# Autodesk Inventor assembly: Stadio7
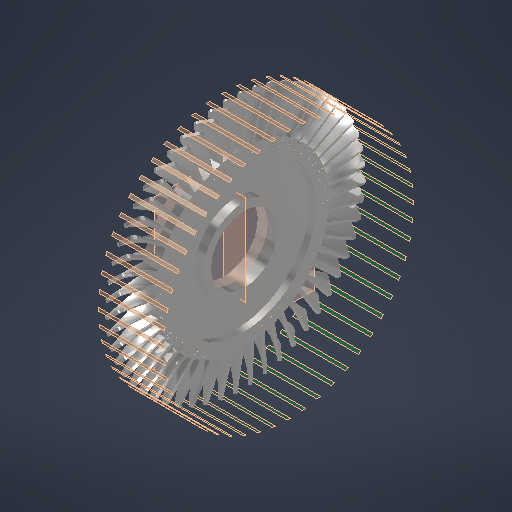
[picture p0: Inventor's stored thumbnail of the model, 512x512]
Saved by Autodesk Inventor 2026.2 (Build 302298010, 298A)
## iProperties
Created: 2026-04-24
Part Number: Stadio7
Document SubType Name: Assembly
Designer: Yan
Author: Yan
## Documents named in this file (3)
- C:\Users\Yan\Desktop\Turbina\Stadio7.iam
- C:\Users\Yan\Desktop\Turbina\DiscoPaleStadio7-DimensioniAprossimate .ipt
- C:\Users\Yan\Desktop\Turbina\PalaStadio7.ipt
## Components (53 placed, 2 different names)
1. DiscoPaleStadio7-DimensioniAprossimate :1 — Mate:1, Mate:2, Mate:3, Mate:4, Mate:5, Mate:6, Mate:7, Mate:8, Mate:9, Mate:10, Mate:11, Mate:12, Mate:13, Mate:14, Mate:15, Mate:16, Mate:17, Mate:18, Mate:19, Mate:20, Mate:21, Mate:22, Mate:23, Mate:24, Mate:25, Mate:26, Mate:27, Mate:28, Mate:29, Mate:30, Mate:31, Mate:32, Mate:33, Mate:34, Mate:35, Mate:36, Mate:37, Mate:38, Mate:39, Mate:40, Mate:41, Mate:42, Mate:43, Mate:44, Mate:45, Mate:46, Mate:47, Mate:48, Mate:49, Mate:50, Mate:51, Mate:52, Mate:53, Mate:54, Mate:55, Mate:56, Mate:57, Mate:58, Mate:59, Mate:60, Mate:61, Mate:62, Mate:63, Mate:64, Mate:65, Mate:66, Mate:67, Mate:68, Mate:69, Mate:70, Mate:71, Mate:72, Mate:73, Mate:74, Mate:75, Mate:76, Mate:77, Mate:78, Mate:79, Mate:80, Mate:81, Mate:82, Mate:83, Mate:84, Mate:85, Mate:86, Mate:87, Mate:88, Mate:89, Mate:90, Mate:91, Mate:92, Mate:93, Mate:94, Mate:95, Mate:96, Mate:97, Mate:98, Mate:99, Mate:100, Mate:101, Mate:102, Mate:103, Flush:1, Flush:2, Flush:3, Flush:4, Flush:5, Flush:6, Flush:7, Flush:8, Flush:9, Flush:10, Flush:11, Flush:12, Flush:13, Flush:14, Flush:15, Flush:16, Flush:17, Flush:18, Flush:19, Flush:20, Flush:21, Flush:22, Flush:23, Flush:24, Flush:25, Flush:26, Flush:27, Flush:28, Flush:29, Flush:30, Flush:31, Flush:32, Flush:33, Flush:34, Flush:35, Flush:36, Flush:37, Flush:38, Flush:39, Flush:40, Flush:41, Flush:42, Flush:43, Flush:44, Flush:45, Flush:46, Flush:47, Flush:48, Flush:49, Flush:50, Flush:51, Flush:52
2. PalaStadio7:1 — Mate:1, Mate:28, Flush:11
3. PalaStadio7:2 — Mate:2, Mate:27, Flush:12
4. PalaStadio7:3 — Mate:3, Mate:29, Flush:13
5. PalaStadio7:4 — Mate:4, Mate:30, Flush:14
6. PalaStadio7:5 — Mate:5, Mate:31, Flush:15
7. PalaStadio7:6 — Mate:6, Mate:32, Flush:16
8. PalaStadio7:7 — Mate:7, Mate:33, Flush:17
9. PalaStadio7:8 — Mate:8, Mate:34, Flush:18
10. PalaStadio7:9 — Mate:9, Mate:35, Flush:19
11. PalaStadio7:10 — Mate:10, Mate:36, Flush:20
12. PalaStadio7:11 — Mate:20, Mate:44, Flush:30
13. PalaStadio7:12 — Mate:19, Mate:48, Flush:29
14. PalaStadio7:13 — Mate:18, Mate:43, Flush:28
15. PalaStadio7:14 — Mate:17, Mate:42, Flush:27
16. PalaStadio7:15 — Mate:16, Mate:41, Flush:26
17. PalaStadio7:16 — Mate:15, Mate:49, Flush:25
18. PalaStadio7:17 — Mate:14, Mate:40, Flush:24
19. PalaStadio7:18 — Mate:13, Mate:39, Flush:23
20. PalaStadio7:19 — Mate:12, Mate:38, Flush:22
21. PalaStadio7:20 — Mate:11, Mate:37, Flush:21
22. PalaStadio7:21 — Mate:56, Mate:64, Flush:41
23. PalaStadio7:22 — Mate:55, Mate:63, Flush:40
24. PalaStadio7:23 — Mate:54, Mate:62, Flush:39
25. PalaStadio7:24 — Mate:53, Mate:61, Flush:37
26. PalaStadio7:25 — Mate:26, Mate:52, Flush:36
27. PalaStadio7:26 — Mate:25, Mate:51, Flush:35
28. PalaStadio7:27 — Mate:24, Mate:50, Flush:34
29. PalaStadio7:28 — Mate:23, Mate:47, Flush:33
30. PalaStadio7:29 — Mate:22, Mate:46, Flush:32
31. PalaStadio7:30 — Mate:21, Mate:45, Flush:31
32. PalaStadio7:31 — Mate:74, Mate:81, Flush:51
33. PalaStadio7:32 — Mate:73, Flush:50
34. PalaStadio7:33 — Mate:72, Mate:80, Flush:49
35. PalaStadio7:34 — Mate:71, Mate:79, Flush:48
36. PalaStadio7:35 — Mate:70, Mate:78, Flush:47
37. PalaStadio7:36 — Mate:69, Mate:77, Flush:46
38. PalaStadio7:37 — Mate:60, Mate:68, Flush:45
39. PalaStadio7:38 — Mate:59, Mate:67, Flush:44
40. PalaStadio7:39 — Mate:58, Mate:66, Flush:43
41. PalaStadio7:40 — Mate:57, Mate:65, Flush:42
42. PalaStadio7:41 — Mate:90, Mate:95, Flush:8
43. PalaStadio7:42 — Mate:89, Mate:96, Flush:7
44. PalaStadio7:43 — Mate:88, Mate:97, Flush:6
45. PalaStadio7:44 — Mate:87, Mate:98, Flush:5
46. PalaStadio7:45 — Mate:86, Mate:99, Flush:4
47. PalaStadio7:46 — Mate:85, Mate:100, Flush:3
48. PalaStadio7:47 — Mate:84, Mate:101, Flush:2
49. PalaStadio7:48 — Mate:83, Mate:102, Flush:1
50. PalaStadio7:49 — Mate:82, Mate:103, Flush:52
51. PalaStadio7:50 — Mate:75, Mate:76, Flush:38
52. PalaStadio7:51 — Mate:92, Mate:93, Flush:10
53. PalaStadio7:52 — Mate:91, Mate:94, Flush:9
## Relationships (155: Mate 103, Flush 52)
- Mate:1: DiscoPaleStadio7-DimensioniAprossimate :1 ↔ PalaStadio7:1
- Mate:2: DiscoPaleStadio7-DimensioniAprossimate :1 ↔ PalaStadio7:2
- Mate:3: DiscoPaleStadio7-DimensioniAprossimate :1 ↔ PalaStadio7:3
- Mate:4: DiscoPaleStadio7-DimensioniAprossimate :1 ↔ PalaStadio7:4
- Mate:5: DiscoPaleStadio7-DimensioniAprossimate :1 ↔ PalaStadio7:5
- Mate:6: DiscoPaleStadio7-DimensioniAprossimate :1 ↔ PalaStadio7:6
- Mate:7: DiscoPaleStadio7-DimensioniAprossimate :1 ↔ PalaStadio7:7
- Mate:8: DiscoPaleStadio7-DimensioniAprossimate :1 ↔ PalaStadio7:8
- Mate:9: DiscoPaleStadio7-DimensioniAprossimate :1 ↔ PalaStadio7:9
- Mate:10: DiscoPaleStadio7-DimensioniAprossimate :1 ↔ PalaStadio7:10
- Mate:11: DiscoPaleStadio7-DimensioniAprossimate :1 ↔ PalaStadio7:20
- Mate:12: DiscoPaleStadio7-DimensioniAprossimate :1 ↔ PalaStadio7:19
- Mate:13: DiscoPaleStadio7-DimensioniAprossimate :1 ↔ PalaStadio7:18
- Mate:14: DiscoPaleStadio7-DimensioniAprossimate :1 ↔ PalaStadio7:17
- Mate:15: DiscoPaleStadio7-DimensioniAprossimate :1 ↔ PalaStadio7:16
- Mate:16: DiscoPaleStadio7-DimensioniAprossimate :1 ↔ PalaStadio7:15
- Mate:17: DiscoPaleStadio7-DimensioniAprossimate :1 ↔ PalaStadio7:14
- Mate:18: DiscoPaleStadio7-DimensioniAprossimate :1 ↔ PalaStadio7:13
- Mate:19: DiscoPaleStadio7-DimensioniAprossimate :1 ↔ PalaStadio7:12
- Mate:20: DiscoPaleStadio7-DimensioniAprossimate :1 ↔ PalaStadio7:11
- Mate:21: DiscoPaleStadio7-DimensioniAprossimate :1 ↔ PalaStadio7:30
- Mate:22: DiscoPaleStadio7-DimensioniAprossimate :1 ↔ PalaStadio7:29
- Mate:23: DiscoPaleStadio7-DimensioniAprossimate :1 ↔ PalaStadio7:28
- Mate:24: DiscoPaleStadio7-DimensioniAprossimate :1 ↔ PalaStadio7:27
- Mate:25: DiscoPaleStadio7-DimensioniAprossimate :1 ↔ PalaStadio7:26
- Mate:26: DiscoPaleStadio7-DimensioniAprossimate :1 ↔ PalaStadio7:25
- Mate:27: DiscoPaleStadio7-DimensioniAprossimate :1 ↔ PalaStadio7:2
- Mate:28: DiscoPaleStadio7-DimensioniAprossimate :1 ↔ PalaStadio7:1
- Mate:29: DiscoPaleStadio7-DimensioniAprossimate :1 ↔ PalaStadio7:3
- Mate:30: DiscoPaleStadio7-DimensioniAprossimate :1 ↔ PalaStadio7:4
- Mate:31: DiscoPaleStadio7-DimensioniAprossimate :1 ↔ PalaStadio7:5
- Mate:32: DiscoPaleStadio7-DimensioniAprossimate :1 ↔ PalaStadio7:6
- Mate:33: DiscoPaleStadio7-DimensioniAprossimate :1 ↔ PalaStadio7:7
- Mate:34: DiscoPaleStadio7-DimensioniAprossimate :1 ↔ PalaStadio7:8
- Mate:35: DiscoPaleStadio7-DimensioniAprossimate :1 ↔ PalaStadio7:9
- Mate:36: DiscoPaleStadio7-DimensioniAprossimate :1 ↔ PalaStadio7:10
- Mate:37: DiscoPaleStadio7-DimensioniAprossimate :1 ↔ PalaStadio7:20
- Mate:38: DiscoPaleStadio7-DimensioniAprossimate :1 ↔ PalaStadio7:19
- Mate:39: DiscoPaleStadio7-DimensioniAprossimate :1 ↔ PalaStadio7:18
- Mate:40: DiscoPaleStadio7-DimensioniAprossimate :1 ↔ PalaStadio7:17
- Mate:41: DiscoPaleStadio7-DimensioniAprossimate :1 ↔ PalaStadio7:15
- Mate:42: DiscoPaleStadio7-DimensioniAprossimate :1 ↔ PalaStadio7:14
- Mate:43: DiscoPaleStadio7-DimensioniAprossimate :1 ↔ PalaStadio7:13
- Mate:44: DiscoPaleStadio7-DimensioniAprossimate :1 ↔ PalaStadio7:11
- Mate:45: DiscoPaleStadio7-DimensioniAprossimate :1 ↔ PalaStadio7:30
- Mate:46: DiscoPaleStadio7-DimensioniAprossimate :1 ↔ PalaStadio7:29
- Mate:47: DiscoPaleStadio7-DimensioniAprossimate :1 ↔ PalaStadio7:28
- Mate:48: DiscoPaleStadio7-DimensioniAprossimate :1 ↔ PalaStadio7:12
- Mate:49: DiscoPaleStadio7-DimensioniAprossimate :1 ↔ PalaStadio7:16
- Mate:50: DiscoPaleStadio7-DimensioniAprossimate :1 ↔ PalaStadio7:27
- Mate:51: DiscoPaleStadio7-DimensioniAprossimate :1 ↔ PalaStadio7:26
- Mate:52: DiscoPaleStadio7-DimensioniAprossimate :1 ↔ PalaStadio7:25
- Mate:53: DiscoPaleStadio7-DimensioniAprossimate :1 ↔ PalaStadio7:24
- Mate:54: DiscoPaleStadio7-DimensioniAprossimate :1 ↔ PalaStadio7:23
- Mate:55: DiscoPaleStadio7-DimensioniAprossimate :1 ↔ PalaStadio7:22
- Mate:56: DiscoPaleStadio7-DimensioniAprossimate :1 ↔ PalaStadio7:21
- Mate:57: DiscoPaleStadio7-DimensioniAprossimate :1 ↔ PalaStadio7:40
- Mate:58: DiscoPaleStadio7-DimensioniAprossimate :1 ↔ PalaStadio7:39
- Mate:59: DiscoPaleStadio7-DimensioniAprossimate :1 ↔ PalaStadio7:38
- Mate:60: DiscoPaleStadio7-DimensioniAprossimate :1 ↔ PalaStadio7:37
- Mate:61: DiscoPaleStadio7-DimensioniAprossimate :1 ↔ PalaStadio7:24
- Mate:62: DiscoPaleStadio7-DimensioniAprossimate :1 ↔ PalaStadio7:23
- Mate:63: DiscoPaleStadio7-DimensioniAprossimate :1 ↔ PalaStadio7:22
- Mate:64: DiscoPaleStadio7-DimensioniAprossimate :1 ↔ PalaStadio7:21
- Mate:65: DiscoPaleStadio7-DimensioniAprossimate :1 ↔ PalaStadio7:40
- Mate:66: DiscoPaleStadio7-DimensioniAprossimate :1 ↔ PalaStadio7:39
- Mate:67: DiscoPaleStadio7-DimensioniAprossimate :1 ↔ PalaStadio7:38
- Mate:68: DiscoPaleStadio7-DimensioniAprossimate :1 ↔ PalaStadio7:37
- Mate:69: DiscoPaleStadio7-DimensioniAprossimate :1 ↔ PalaStadio7:36
- Mate:70: DiscoPaleStadio7-DimensioniAprossimate :1 ↔ PalaStadio7:35
- Mate:71: DiscoPaleStadio7-DimensioniAprossimate :1 ↔ PalaStadio7:34
- Mate:72: DiscoPaleStadio7-DimensioniAprossimate :1 ↔ PalaStadio7:33
- Mate:73: DiscoPaleStadio7-DimensioniAprossimate :1 ↔ PalaStadio7:32
- Mate:74: DiscoPaleStadio7-DimensioniAprossimate :1 ↔ PalaStadio7:31
- Mate:75: DiscoPaleStadio7-DimensioniAprossimate :1 ↔ PalaStadio7:50
- Mate:76: DiscoPaleStadio7-DimensioniAprossimate :1 ↔ PalaStadio7:50
- Mate:77: DiscoPaleStadio7-DimensioniAprossimate :1 ↔ PalaStadio7:36
- Mate:78: DiscoPaleStadio7-DimensioniAprossimate :1 ↔ PalaStadio7:35
- Mate:79: DiscoPaleStadio7-DimensioniAprossimate :1 ↔ PalaStadio7:34
- Mate:80: DiscoPaleStadio7-DimensioniAprossimate :1 ↔ PalaStadio7:33
- Mate:81: DiscoPaleStadio7-DimensioniAprossimate :1 ↔ PalaStadio7:31
- Mate:82: DiscoPaleStadio7-DimensioniAprossimate :1 ↔ PalaStadio7:49
- Mate:83: DiscoPaleStadio7-DimensioniAprossimate :1 ↔ PalaStadio7:48
- Mate:84: DiscoPaleStadio7-DimensioniAprossimate :1 ↔ PalaStadio7:47
- Mate:85: DiscoPaleStadio7-DimensioniAprossimate :1 ↔ PalaStadio7:46
- Mate:86: DiscoPaleStadio7-DimensioniAprossimate :1 ↔ PalaStadio7:45
- Mate:87: DiscoPaleStadio7-DimensioniAprossimate :1 ↔ PalaStadio7:44
- Mate:88: DiscoPaleStadio7-DimensioniAprossimate :1 ↔ PalaStadio7:43
- Mate:89: DiscoPaleStadio7-DimensioniAprossimate :1 ↔ PalaStadio7:42
- Mate:90: DiscoPaleStadio7-DimensioniAprossimate :1 ↔ PalaStadio7:41
- Mate:91: DiscoPaleStadio7-DimensioniAprossimate :1 ↔ PalaStadio7:52
- Mate:92: DiscoPaleStadio7-DimensioniAprossimate :1 ↔ PalaStadio7:51
- Mate:93: DiscoPaleStadio7-DimensioniAprossimate :1 ↔ PalaStadio7:51
- Mate:94: DiscoPaleStadio7-DimensioniAprossimate :1 ↔ PalaStadio7:52
- Mate:95: DiscoPaleStadio7-DimensioniAprossimate :1 ↔ PalaStadio7:41
- Mate:96: DiscoPaleStadio7-DimensioniAprossimate :1 ↔ PalaStadio7:42
- Mate:97: DiscoPaleStadio7-DimensioniAprossimate :1 ↔ PalaStadio7:43
- Mate:98: DiscoPaleStadio7-DimensioniAprossimate :1 ↔ PalaStadio7:44
- Mate:99: DiscoPaleStadio7-DimensioniAprossimate :1 ↔ PalaStadio7:45
- Mate:100: DiscoPaleStadio7-DimensioniAprossimate :1 ↔ PalaStadio7:46
- Mate:101: DiscoPaleStadio7-DimensioniAprossimate :1 ↔ PalaStadio7:47
- Mate:102: DiscoPaleStadio7-DimensioniAprossimate :1 ↔ PalaStadio7:48
- Mate:103: DiscoPaleStadio7-DimensioniAprossimate :1 ↔ PalaStadio7:49
- Flush:1: DiscoPaleStadio7-DimensioniAprossimate :1 ↔ PalaStadio7:48
- Flush:2: DiscoPaleStadio7-DimensioniAprossimate :1 ↔ PalaStadio7:47
- Flush:3: DiscoPaleStadio7-DimensioniAprossimate :1 ↔ PalaStadio7:46
- Flush:4: DiscoPaleStadio7-DimensioniAprossimate :1 ↔ PalaStadio7:45
- Flush:5: DiscoPaleStadio7-DimensioniAprossimate :1 ↔ PalaStadio7:44
- Flush:6: DiscoPaleStadio7-DimensioniAprossimate :1 ↔ PalaStadio7:43
- Flush:7: DiscoPaleStadio7-DimensioniAprossimate :1 ↔ PalaStadio7:42
- Flush:8: DiscoPaleStadio7-DimensioniAprossimate :1 ↔ PalaStadio7:41
- Flush:9: DiscoPaleStadio7-DimensioniAprossimate :1 ↔ PalaStadio7:52
- Flush:10: DiscoPaleStadio7-DimensioniAprossimate :1 ↔ PalaStadio7:51
- Flush:11: DiscoPaleStadio7-DimensioniAprossimate :1 ↔ PalaStadio7:1
- Flush:12: DiscoPaleStadio7-DimensioniAprossimate :1 ↔ PalaStadio7:2
- Flush:13: DiscoPaleStadio7-DimensioniAprossimate :1 ↔ PalaStadio7:3
- Flush:14: DiscoPaleStadio7-DimensioniAprossimate :1 ↔ PalaStadio7:4
- Flush:15: DiscoPaleStadio7-DimensioniAprossimate :1 ↔ PalaStadio7:5
- Flush:16: DiscoPaleStadio7-DimensioniAprossimate :1 ↔ PalaStadio7:6
- Flush:17: DiscoPaleStadio7-DimensioniAprossimate :1 ↔ PalaStadio7:7
- Flush:18: DiscoPaleStadio7-DimensioniAprossimate :1 ↔ PalaStadio7:8
- Flush:19: DiscoPaleStadio7-DimensioniAprossimate :1 ↔ PalaStadio7:9
- Flush:20: DiscoPaleStadio7-DimensioniAprossimate :1 ↔ PalaStadio7:10
- Flush:21: DiscoPaleStadio7-DimensioniAprossimate :1 ↔ PalaStadio7:20
- Flush:22: DiscoPaleStadio7-DimensioniAprossimate :1 ↔ PalaStadio7:19
- Flush:23: DiscoPaleStadio7-DimensioniAprossimate :1 ↔ PalaStadio7:18
- Flush:24: DiscoPaleStadio7-DimensioniAprossimate :1 ↔ PalaStadio7:17
- Flush:25: DiscoPaleStadio7-DimensioniAprossimate :1 ↔ PalaStadio7:16
- Flush:26: DiscoPaleStadio7-DimensioniAprossimate :1 ↔ PalaStadio7:15
- Flush:27: DiscoPaleStadio7-DimensioniAprossimate :1 ↔ PalaStadio7:14
- Flush:28: DiscoPaleStadio7-DimensioniAprossimate :1 ↔ PalaStadio7:13
- Flush:29: DiscoPaleStadio7-DimensioniAprossimate :1 ↔ PalaStadio7:12
- Flush:30: DiscoPaleStadio7-DimensioniAprossimate :1 ↔ PalaStadio7:11
- Flush:31: DiscoPaleStadio7-DimensioniAprossimate :1 ↔ PalaStadio7:30
- Flush:32: DiscoPaleStadio7-DimensioniAprossimate :1 ↔ PalaStadio7:29
- Flush:33: DiscoPaleStadio7-DimensioniAprossimate :1 ↔ PalaStadio7:28
- Flush:34: DiscoPaleStadio7-DimensioniAprossimate :1 ↔ PalaStadio7:27
- Flush:35: DiscoPaleStadio7-DimensioniAprossimate :1 ↔ PalaStadio7:26
- Flush:36: DiscoPaleStadio7-DimensioniAprossimate :1 ↔ PalaStadio7:25
- Flush:37: DiscoPaleStadio7-DimensioniAprossimate :1 ↔ PalaStadio7:24
- Flush:38: DiscoPaleStadio7-DimensioniAprossimate :1 ↔ PalaStadio7:50
- Flush:39: DiscoPaleStadio7-DimensioniAprossimate :1 ↔ PalaStadio7:23
- Flush:40: DiscoPaleStadio7-DimensioniAprossimate :1 ↔ PalaStadio7:22
- Flush:41: DiscoPaleStadio7-DimensioniAprossimate :1 ↔ PalaStadio7:21
- Flush:42: DiscoPaleStadio7-DimensioniAprossimate :1 ↔ PalaStadio7:40
- Flush:43: DiscoPaleStadio7-DimensioniAprossimate :1 ↔ PalaStadio7:39
- Flush:44: DiscoPaleStadio7-DimensioniAprossimate :1 ↔ PalaStadio7:38
- Flush:45: DiscoPaleStadio7-DimensioniAprossimate :1 ↔ PalaStadio7:37
- Flush:46: DiscoPaleStadio7-DimensioniAprossimate :1 ↔ PalaStadio7:36
- Flush:47: DiscoPaleStadio7-DimensioniAprossimate :1 ↔ PalaStadio7:35
- Flush:48: DiscoPaleStadio7-DimensioniAprossimate :1 ↔ PalaStadio7:34
- Flush:49: DiscoPaleStadio7-DimensioniAprossimate :1 ↔ PalaStadio7:33
- Flush:50: DiscoPaleStadio7-DimensioniAprossimate :1 ↔ PalaStadio7:32
- Flush:51: DiscoPaleStadio7-DimensioniAprossimate :1 ↔ PalaStadio7:31
- Flush:52: DiscoPaleStadio7-DimensioniAprossimate :1 ↔ PalaStadio7:49
